# Autodesk Inventor assembly: Assembled Tall Chassis
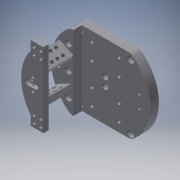
[picture p0: Inventor's stored thumbnail of the model, 180x180]
Saved by Autodesk Inventor 2016 (Build 200138000, 138)
## iProperties
Created: 2017-03-17
Part Number: Assembled Tall Chassis
Document SubType Name: Assembly
Designer: Billy
Author: Billy
## Documents named in this file (3)
- C:\Users\billy_000\Documents\Micromouse\Official\MicroMouse2017\CAD\Assembled Tall Chassis.iam
- C:\Users\billy_000\Documents\Micromouse\Official\MicroMouse2017\CAD\Modular Chassis (Tall).ipt
- C:\Users\billy_000\Documents\Micromouse\Official\MicroMouse2017\CAD\Sensor Shield.ipt
## Components (2 placed, 2 different names)
1. Modular Chassis (Tall):1 — Insert:1, Insert:2
2. Sensor Shield:1 — Insert:1, Insert:2
## Relationships (2: Insert 2)
- Insert:1: Modular Chassis (Tall):1 ↔ Sensor Shield:1
- Insert:2: Modular Chassis (Tall):1 ↔ Sensor Shield:1
